# Autodesk Inventor assembly: robot
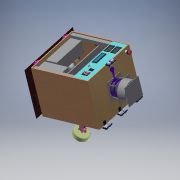
[picture p0: Inventor's stored thumbnail of the model, 180x180]
Saved by Autodesk Inventor 2019 (Build 230136000, 136)
## iProperties
Created: 2019-03-18
Part Number: robot
Document SubType Name: Assembly
Designer: franc
Mass: 1757.08 g
Surface Area: 9591.54 cm^2
Volume: 1726.16 cm^3
Density: 1.01791 g/cm^3
Author: franc
## Documents named in this file (15)
- C:\Users\franc\Desktop\EsialRobotik\Mecanique\2019\robot\robot.iam
- C:\Users\franc\Desktop\EsialRobotik\Mecanique\2019\robot\socle-robot.ipt
- C:\Users\franc\Desktop\EsialRobotik\Mecanique\base_roulante\baseRoulante.iam
- C:\Users\franc\Desktop\EsialRobotik\Mecanique\2019\robot\face-lateral.ipt
- C:\Users\franc\Desktop\EsialRobotik\Mecanique\2019\robot\profile_alu.ipt
- C:\Users\franc\Desktop\EsialRobotik\Mecanique\2019\robot\support_arriere.iam
- C:\Users\franc\Desktop\EsialRobotik\Mecanique\2019\robot\toit.iam
- C:\Users\franc\Desktop\EsialRobotik\Mecanique\composants\Profile\equerreEtage.ipt
- C:\Users\franc\Desktop\EsialRobotik\Mecanique\composants\Profile\calle.iam
- C:\Users\franc\Desktop\EsialRobotik\Mecanique\composants\SRF04\SRF04_sur_support.iam
- C:\Users\franc\Desktop\EsialRobotik\Mecanique\2019\robot\bras\bras.iam
- C:\Users\franc\Desktop\EsialRobotik\Mecanique\2019\robot\palet.ipt
- C:\Users\franc\Desktop\EsialRobotik\Mecanique\composants\Batterie\grosse-batterie.ipt
- C:\Users\franc\Desktop\EsialRobotik\Mecanique\composants\Batterie\petite-batterie.ipt
- C:\Users\franc\Desktop\EsialRobotik\Mecanique\2019\robot\étage.iam
## Components (32 placed, 14 different names)
1. socle-robot:1 — Mate:1, Mate:3, Placage:4, Affleurement:1, Affleurement:2, Placage:5, Affleurement:3, Affleurement:4, Placage:10, Placage:11, Placage:12, Placage:13, Placage:17, Placage:18, Placage:19, Placage:20, Placage:26, Placage:27, Placage:28, Placage:29, Affleurement:15, Affleurement:16, Affleurement:17, Affleurement:18, Affleurement:19, Affleurement:20, Affleurement:21, Affleurement:22, Placage:38, Placage:39, Placage:40, Placage:41, Affleurement:25, Affleurement:26, Affleurement:27, Affleurement:28, Placage:42, Affleurement:29, Placage:43, Affleurement:30, Placage:45, Placage:48, Placage:52, Placage:53, Placage:60
2. baseRoulante:1 [sub-assembly] — Mate:1, Mate:3, Placage:60
3. face-lateral:1 — Placage:4, Affleurement:1, Affleurement:2, Placage:6, Placage:7, Affleurement:6, Affleurement:8, Placage:46, Placage:49
4. face-lateral:2 — Placage:5, Affleurement:3, Affleurement:4, Placage:8, Placage:9, Affleurement:5, Affleurement:7, Placage:15, Placage:16, Affleurement:9, Affleurement:10
5. profile_alu:1 — Placage:6, Placage:10, Affleurement:8, Placage:25, Affleurement:14, Placage:44, Placage:47, Placage:54
6. profile_alu:2 — Placage:7, Placage:11, Affleurement:6, Placage:22, Affleurement:12
7. profile_alu:3 — Placage:9, Placage:13, Affleurement:7, Placage:14, Placage:24, Affleurement:13, Placage:55
8. profile_alu:4 — Placage:8, Placage:12, Affleurement:5, Placage:21, Affleurement:11
9. support_arriere:1 [sub-assembly] — Placage:14, Placage:15, Placage:23
10. toit:1 [sub-assembly] — Placage:16, Affleurement:9, Affleurement:10, Placage:23, Placage:30, Placage:31, Placage:32, Placage:33, Placage:34, Angle:1, Placage:35, Placage:36, Placage:37, Angle:2, Angle:3, Angle:4
11. equerreEtage:1 — Placage:17, Placage:21, Affleurement:11
12. equerreEtage:2 — Placage:18, Placage:22, Affleurement:12
13. equerreEtage:3 — Placage:19, Placage:24, Affleurement:13
14. equerreEtage:4 — Placage:20, Placage:25, Affleurement:14
15. calle:1 [sub-assembly] — Placage:29, Affleurement:18, Affleurement:19
16. calle:2 [sub-assembly] — Placage:28, Affleurement:16, Affleurement:20
17. calle:3 [sub-assembly] — Placage:27, Affleurement:15, Affleurement:22
18. calle:4 [sub-assembly] — Placage:26, Affleurement:17, Affleurement:21
19. SRF04_sur_support:1 [sub-assembly] — Placage:33, Placage:34, Angle:1
20. SRF04_sur_support:2 [sub-assembly] — Placage:31, Placage:36, Angle:3
21. SRF04_sur_support:3 [sub-assembly] — Placage:30, Placage:35, Angle:4
22. SRF04_sur_support:4 [sub-assembly] — Placage:32, Placage:37, Angle:2
23. bras:1 [sub-assembly] — Placage:38, Affleurement:25, Affleurement:28, Placage:51, Placage:56, Placage:57
24. bras:2 [sub-assembly] — Placage:39, Affleurement:26, Affleurement:27, Placage:50, Placage:58, Placage:59
25. palet:1 — Placage:40, Placage:51, Placage:53
26. palet:2 — Placage:41, Placage:50, Placage:52
27. grosse-batterie:1 — Placage:42, Affleurement:29, Placage:55
28. petite-batterie:1 — Placage:43, Affleurement:30, Placage:54
29. étage:1 [sub-assembly] — Placage:44, Placage:45, Placage:46
30. étage:2 [sub-assembly] — Placage:47, Placage:48, Placage:49
31. palet:3 — Placage:56, Placage:57
32. palet:4 — Placage:58, Placage:59
## Relationships (91: Mate 59, Flush 28, Angle 4)
- Mate:1: socle-robot:1 ↔ baseRoulante:1
- Mate:3: socle-robot:1 ↔ baseRoulante:1
- Placage:4 [Mate]: socle-robot:1 ↔ face-lateral:1
- Affleurement:1 [Flush]: socle-robot:1 ↔ face-lateral:1
- Affleurement:2 [Flush]: socle-robot:1 ↔ face-lateral:1
- Placage:5 [Mate]: socle-robot:1 ↔ face-lateral:2
- Affleurement:3 [Flush]: socle-robot:1 ↔ face-lateral:2
- Affleurement:4 [Flush]: socle-robot:1 ↔ face-lateral:2
- Placage:6 [Mate]: face-lateral:1 ↔ profile_alu:1
- Placage:7 [Mate]: face-lateral:1 ↔ profile_alu:2
- Placage:8 [Mate]: face-lateral:2 ↔ profile_alu:4
- Placage:9 [Mate]: face-lateral:2 ↔ profile_alu:3
- Placage:10 [Mate]: socle-robot:1 ↔ profile_alu:1
- Placage:11 [Mate]: socle-robot:1 ↔ profile_alu:2
- Placage:12 [Mate]: socle-robot:1 ↔ profile_alu:4
- Placage:13 [Mate]: socle-robot:1 ↔ profile_alu:3
- Affleurement:5 [Flush]: face-lateral:2 ↔ profile_alu:4
- Affleurement:6 [Flush]: face-lateral:1 ↔ profile_alu:2
- Affleurement:7 [Flush] (5 mm): face-lateral:2 ↔ profile_alu:3
- Affleurement:8 [Flush] (5 mm): face-lateral:1 ↔ profile_alu:1
- Placage:14 [Mate]: profile_alu:3 ↔ support_arriere:1
- Placage:15 [Mate]: face-lateral:2 ↔ support_arriere:1
- Placage:16 [Mate]: face-lateral:2 ↔ toit:1
- Affleurement:9 [Flush]: face-lateral:2 ↔ toit:1
- Affleurement:10 [Flush]: face-lateral:2 ↔ toit:1
- Placage:17 [Mate]: socle-robot:1 ↔ equerreEtage:1
- Placage:18 [Mate]: socle-robot:1 ↔ equerreEtage:2
- Placage:19 [Mate]: socle-robot:1 ↔ equerreEtage:3
- Placage:20 [Mate]: socle-robot:1 ↔ equerreEtage:4
- Placage:21 [Mate]: profile_alu:4 ↔ equerreEtage:1
- Affleurement:11 [Flush]: profile_alu:4 ↔ equerreEtage:1
- Placage:22 [Mate]: profile_alu:2 ↔ equerreEtage:2
- Affleurement:12 [Flush]: profile_alu:2 ↔ equerreEtage:2
- Placage:23 [Mate]: support_arriere:1 ↔ toit:1
- Placage:24 [Mate]: profile_alu:3 ↔ equerreEtage:3
- Affleurement:13 [Flush]: profile_alu:3 ↔ equerreEtage:3
- Placage:25 [Mate]: profile_alu:1 ↔ equerreEtage:4
- Affleurement:14 [Flush]: profile_alu:1 ↔ equerreEtage:4
- Placage:26 [Mate]: socle-robot:1 ↔ calle:4
- Placage:27 [Mate]: socle-robot:1 ↔ calle:3
- Placage:28 [Mate]: socle-robot:1 ↔ calle:2
- Placage:29 [Mate]: socle-robot:1 ↔ calle:1
- Affleurement:15 [Flush]: socle-robot:1 ↔ calle:3
- Affleurement:16 [Flush]: socle-robot:1 ↔ calle:2
- Affleurement:17 [Flush]: socle-robot:1 ↔ calle:4
- Affleurement:18 [Flush]: socle-robot:1 ↔ calle:1
- Affleurement:19 [Flush] (30 mm): socle-robot:1 ↔ calle:1
- Affleurement:20 [Flush] (30 mm): socle-robot:1 ↔ calle:2
- Affleurement:21 [Flush] (30 mm): socle-robot:1 ↔ calle:4
- Affleurement:22 [Flush] (30 mm): socle-robot:1 ↔ calle:3
- Placage:30 [Mate]: toit:1 ↔ SRF04_sur_support:3
- Placage:31 [Mate]: toit:1 ↔ SRF04_sur_support:2
- Placage:32 [Mate]: toit:1 ↔ SRF04_sur_support:4
- Placage:33 [Mate]: toit:1 ↔ SRF04_sur_support:1
- Placage:34 [Mate]: toit:1 ↔ SRF04_sur_support:1
- Angle:1 (0 deg): toit:1 ↔ SRF04_sur_support:1
- Placage:35 [Mate]: toit:1 ↔ SRF04_sur_support:3
- Placage:36 [Mate]: toit:1 ↔ SRF04_sur_support:2
- Placage:37 [Mate]: toit:1 ↔ SRF04_sur_support:4
- Angle:2 (0 deg): toit:1 ↔ SRF04_sur_support:4
- Angle:3 (0 deg): toit:1 ↔ SRF04_sur_support:2
- Angle:4 (0 deg): toit:1 ↔ SRF04_sur_support:3
- Placage:38 [Mate]: socle-robot:1 ↔ bras:1
- Placage:39 [Mate]: socle-robot:1 ↔ bras:2
- Placage:40 [Mate]: socle-robot:1 ↔ palet:1
- Placage:41 [Mate]: socle-robot:1 ↔ palet:2
- Affleurement:25 [Flush] (35 mm): socle-robot:1 ↔ bras:1
- Affleurement:26 [Flush] (35 mm): socle-robot:1 ↔ bras:2
- Affleurement:27 [Flush] (40 mm): socle-robot:1 ↔ bras:2
- Affleurement:28 [Flush] (40 mm): socle-robot:1 ↔ bras:1
- Placage:42 [Mate]: socle-robot:1 ↔ grosse-batterie:1
- Affleurement:29 [Flush] (20 mm): socle-robot:1 ↔ grosse-batterie:1
- Placage:43 [Mate]: socle-robot:1 ↔ petite-batterie:1
- Affleurement:30 [Flush] (-20 mm): socle-robot:1 ↔ petite-batterie:1
- Placage:44 [Mate]: profile_alu:1 ↔ étage:1
- Placage:45 [Mate] (150 mm): socle-robot:1 ↔ étage:1
- Placage:46 [Mate]: face-lateral:1 ↔ étage:1
- Placage:47 [Mate]: profile_alu:1 ↔ étage:2
- Placage:48 [Mate] (225 mm): socle-robot:1 ↔ étage:2
- Placage:49 [Mate]: face-lateral:1 ↔ étage:2
- Placage:50 [Mate] (45 mm): bras:2 ↔ palet:2
- Placage:51 [Mate] (45 mm): bras:1 ↔ palet:1
- Placage:52 [Mate] (-30 mm): socle-robot:1 ↔ palet:2
- Placage:53 [Mate] (-30 mm): socle-robot:1 ↔ palet:1
- Placage:54 [Mate]: profile_alu:1 ↔ petite-batterie:1
- Placage:55 [Mate]: profile_alu:3 ↔ grosse-batterie:1
- Placage:56 [Mate]: bras:1 ↔ palet:3
- Placage:57 [Mate]: bras:1 ↔ palet:3
- Placage:58 [Mate]: bras:2 ↔ palet:4
- Placage:59 [Mate]: bras:2 ↔ palet:4
- Placage:60 [Mate]: socle-robot:1 ↔ baseRoulante:1
